# Autodesk Inventor assembly: HalfChassisAssem
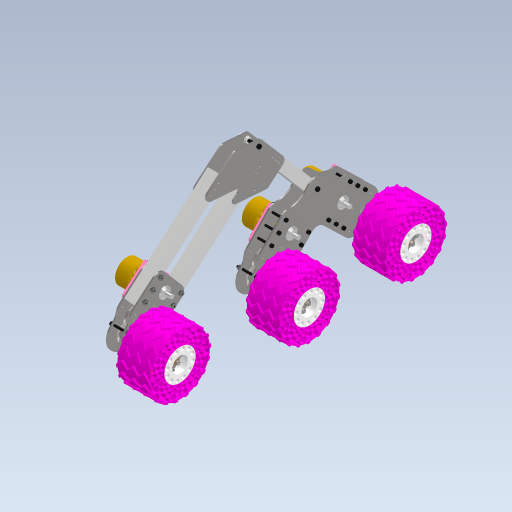
[picture p0: Inventor's stored thumbnail of the model, 512x512]
Saved by Autodesk Inventor 2023 (Build 270158000, 158)
## iProperties
Created: 2023-04-06
Part Number: HalfChassisAssem
Document SubType Name: Assembly
Designer: Dave
Mass: 5362.71 g
Surface Area: 20188.6 cm^2
Volume: 2426.63 cm^3
Density: 2.20995 g/cm^3
Author: Dave
## Documents named in this file (14)
- C:\Users\Dave\Documents\GitHub\BehrendURCMechanical\CAD\Chassis V3\HalfChassisAssem.iam
- C:\Users\Dave\Documents\GitHub\BehrendURCMechanical\CAD\Chassis V3\L3 Gearbox Assembly.iam
- C:\Users\Dave\Documents\GitHub\BehrendURCMechanical\CAD\Chassis V3\L1 Gearbox Assembly.iam
- C:\Users\Dave\Documents\GitHub\BehrendURCMechanical\CAD\Chassis V3\HipPivotPlate.ipt
- C:\Users\Dave\Documents\GitHub\BehrendURCMechanical\CAD\Chassis V3\aluminumextrusiontool.ipt
- C:\Users\Dave\Documents\GitHub\BehrendURCMechanical\CAD\Chassis V3\aluminumextrusiontool\aluminumextrusiontool-17-10.6in.ipt
- C:\Users\Dave\Documents\GitHub\BehrendURCMechanical\CAD\Chassis V3\Wheel\WheelAssembly_v8.iam
- C:\Users\Dave\Documents\GitHub\BehrendURCMechanical\CAD\Chassis V3\aluminumextrusiontool\aluminumextrusiontool-17-13.31255in.ipt
- C:\Users\Dave\Documents\GitHub\BehrendURCMechanical\CAD\Chassis V3\Pivot Files and Assembly\PivotAssembly.iam
- C:\Users\Dave\Documents\GitHub\BehrendURCMechanical\CAD\Chassis V3\aluminumextrusiontool\aluminumextrusiontool-17-7.9.ipt
- C:\Users\Dave\Documents\GitHub\BehrendURCMechanical\CAD\Chassis V3\60645K211_Ball Joint Linkage.ipt
- C:\Users\Dave\Documents\GitHub\BehrendURCMechanical\CAD\Chassis V3\59915K481_Corrosion-Resistant Ball Joint Rod End.ipt
- C:\Users\Dave\Documents\GitHub\BehrendURCMechanical\CAD\Chassis V3\91333A140_Low-Strength Steel Nylon-Insert Locknut.ipt
- C:\Users\Dave\Documents\GitHub\BehrendURCMechanical\CAD\Chassis V3\90107A011_316 Stainless Steel Washer.ipt
## Components (16 placed, 12 different names)
1. L3 Gearbox Assembly:1 [sub-assembly] — Mate:4, Tangent:2, Mate:8, Flush:11, Mate:10, Insert:1, Mate:12
2. L1 Gearbox Assembly:1 [sub-assembly] — Flush:2, Flush:3, Mate:1, Flush:6, Mate:2, Flush:7, Mate:3, Mate:7, Flush:10, Mate:11, Flush:13, Tangent:3
3. HipPivotPlate:1 — Flush:3, Flush:4, Flush:5, Mate:5, Insert:3, Insert:4
4. HipPivotPlate:2 — Flush:2, Flush:4, Flush:5, Mate:1, Flush:6, Mate:4, Flush:8, Tangent:1, Mate:6, Flush:9, Insert:2
5. aluminumextrusiontool-17-10.6in:1 — Mate:2, Flush:7, Mate:3
6. aluminumextrusiontool-17-7.9:2 — Mate:5, Flush:8, Tangent:1, Tangent:2, Mate:10
7. WheelAssembly_v8:1 [sub-assembly] — Mate:7, Flush:10
8. WheelAssembly_v8:2 [sub-assembly] — Mate:8, Flush:11, Flush:14
9. WheelAssembly_v8:3 [sub-assembly] — Flush:14, Mate:12
10. aluminumextrusiontool-17-13.31255in:3 — Mate:11, Flush:13, Tangent:3
11. PivotAssembly:2 [sub-assembly] — Insert:1
12. PivotAssembly:3 [sub-assembly] — Insert:2
13. 60645K211_Ball Joint Linkage:1 — Insert:3, Mate:13
14. 59915K481_Corrosion-Resistant Ball Joint Rod End:1 — Mate:13
15. 91333A140_Low-Strength Steel Nylon-Insert Locknut:1 — Insert:5
16. 90107A011_316 Stainless Steel Washer:1 — Insert:4, Insert:5
## Relationships (32: Flush 12, Mate 12, Insert 5, Tangent 3)
- Flush:2: L1 Gearbox Assembly:1 ↔ HipPivotPlate:2
- Flush:3: L1 Gearbox Assembly:1 ↔ HipPivotPlate:1
- Flush:4: HipPivotPlate:1 ↔ HipPivotPlate:2
- Flush:5: HipPivotPlate:1 ↔ HipPivotPlate:2
- Mate:1 (396 mm): L1 Gearbox Assembly:1 ↔ HipPivotPlate:2
- Flush:6: L1 Gearbox Assembly:1 ↔ HipPivotPlate:2
- Mate:2: L1 Gearbox Assembly:1 ↔ aluminumextrusiontool-17-10.6in:1
- Flush:7: L1 Gearbox Assembly:1 ↔ aluminumextrusiontool-17-10.6in:1
- Mate:3 (-76.2 mm): L1 Gearbox Assembly:1 ↔ aluminumextrusiontool-17-10.6in:1
- Mate:4 (216 mm): L3 Gearbox Assembly:1 ↔ HipPivotPlate:2
- Mate:5: HipPivotPlate:1 ↔ aluminumextrusiontool-17-7.9:2
- Flush:8: HipPivotPlate:2 ↔ aluminumextrusiontool-17-7.9:2
- Tangent:1 (12.7 mm): HipPivotPlate:2 ↔ aluminumextrusiontool-17-7.9:2
- Tangent:2 (6.35 mm): L3 Gearbox Assembly:1 ↔ aluminumextrusiontool-17-7.9:2
- Mate:6: HipPivotPlate:2
- Flush:9: HipPivotPlate:2
- Mate:7: L1 Gearbox Assembly:1 ↔ WheelAssembly_v8:1
- Mate:8: L3 Gearbox Assembly:1 ↔ WheelAssembly_v8:2
- Flush:10: L1 Gearbox Assembly:1 ↔ WheelAssembly_v8:1
- Flush:11: L3 Gearbox Assembly:1 ↔ WheelAssembly_v8:2
- Mate:10: L3 Gearbox Assembly:1 ↔ aluminumextrusiontool-17-7.9:2
- Mate:11: L1 Gearbox Assembly:1 ↔ aluminumextrusiontool-17-13.31255in:3
- Flush:13: L1 Gearbox Assembly:1 ↔ aluminumextrusiontool-17-13.31255in:3
- Tangent:3 (12.7 mm): L1 Gearbox Assembly:1 ↔ aluminumextrusiontool-17-13.31255in:3
- Insert:1: L3 Gearbox Assembly:1 ↔ PivotAssembly:2
- Insert:2: HipPivotPlate:2 ↔ PivotAssembly:3
- Flush:14: WheelAssembly_v8:2 ↔ WheelAssembly_v8:3
- Mate:12: L3 Gearbox Assembly:1 ↔ WheelAssembly_v8:3
- Insert:3: HipPivotPlate:1 ↔ 60645K211_Ball Joint Linkage:1
- Insert:4: HipPivotPlate:1 ↔ 90107A011_316 Stainless Steel Washer:1
- Insert:5: 91333A140_Low-Strength Steel Nylon-Insert Locknut:1 ↔ 90107A011_316 Stainless Steel Washer:1
- Mate:13: 60645K211_Ball Joint Linkage:1 ↔ 59915K481_Corrosion-Resistant Ball Joint Rod End:1
